# Autodesk Inventor assembly: STEEL FRAME ASSY
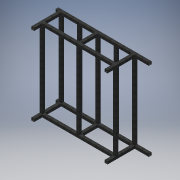
[picture p0: Inventor's stored thumbnail of the model, 180x180]
Saved by Autodesk Inventor 2017 (Build 210142000, 142)
## iProperties
Part Number: STEEL FRAME ASSY
Material: Genérico
Document SubType Name: Assembly
Designer: Cristian
Author: Cristian
## Documents named in this file (6)
- C:\Users\Cristian\Desktop\DISEÑO\FRAME\CNCO 75-3 FRAME\STEEL FRAME ASSY.iam
- C:\Users\Cristian\Desktop\DISEÑO\FRAME\CNCO 75-3 FRAME\2570 STEEL PROFILE.ipt
- C:\Users\Cristian\Desktop\DISEÑO\FRAME\CNCO 75-3 FRAME\2100 STEEL PROFILE.ipt
- C:\Users\Cristian\Desktop\DISEÑO\FRAME\CNCO 75-3 FRAME\450 STEEL PROFILE.ipt
- C:\Users\Cristian\Desktop\DISEÑO\FRAME\CNCO 75-3 FRAME\750 STEEL PROFILE.ipt
- C:\Users\Cristian\Desktop\DISEÑO\FRAME\CNCO 75-3 FRAME\1950 STEEL PROFILE.ipt
## Components (18 placed, 5 different names)
1. 2100 STEEL PROFILE:1 — Coincidencia:1, Coincidencia:2, Coincidencia:3, Coincidencia:4, Nivelación:1, Coincidencia:5, Nivelación:2, Nivelación:3, Nivelación:6, Nivelación:21, Nivelación:23
2. 2570 STEEL PROFILE:1 — Coincidencia:4, Nivelación:1, Coincidencia:6, Nivelación:4, Coincidencia:9, Nivelación:9, Nivelación:10, Coincidencia:16, Nivelación:14, Nivelación:18
3. 2570 STEEL PROFILE:2 — Coincidencia:5, Nivelación:2, Coincidencia:7, Nivelación:5, Coincidencia:8, Nivelación:7, Nivelación:8, Coincidencia:14, Nivelación:13, Coincidencia:18, Nivelación:15, Coincidencia:19, Nivelación:19, Coincidencia:20, Nivelación:22, Coincidencia:21, Nivelación:24
4. 450 STEEL PROFILE:1 — Coincidencia:6, Nivelación:3, Nivelación:4, Coincidencia:13
5. 450 STEEL PROFILE:2 — Coincidencia:7, Nivelación:5, Nivelación:6, Coincidencia:11, Nivelación:31
6. 750 STEEL PROFILE:1 — Coincidencia:16, Nivelación:14, Coincidencia:17
7. 750 STEEL PROFILE:2 — Coincidencia:14, Nivelación:13, Coincidencia:15, Nivelación:20, Coincidencia:23, Nivelación:28
8. 750 STEEL PROFILE:3 — Coincidencia:8, Nivelación:7, Nivelación:8, Coincidencia:10, Nivelación:11, Nivelación:16, Coincidencia:22, Nivelación:27
9. 750 STEEL PROFILE:4 — Coincidencia:9, Nivelación:9, Nivelación:10, Coincidencia:12, Nivelación:12, Nivelación:17
10. 1950 STEEL PROFILE:1 — Coincidencia:10, Nivelación:11, Coincidencia:11, Coincidencia:15, Nivelación:26, Nivelación:29, Coincidencia:24, Nivelación:30
11. 1950 STEEL PROFILE:2 — Coincidencia:12, Nivelación:12, Coincidencia:13, Coincidencia:17
12. 2100 STEEL PROFILE:2 — Coincidencia:21, Nivelación:24, Nivelación:25
13. 2100 STEEL PROFILE:3 — Coincidencia:20, Nivelación:22, Nivelación:23
14. 2100 STEEL PROFILE:4 — Coincidencia:18, Nivelación:15, Nivelación:16, Nivelación:17, Nivelación:18, Nivelación:25
15. 2100 STEEL PROFILE:5 — Coincidencia:19, Nivelación:19, Nivelación:20, Nivelación:21
16. 2100 STEEL PROFILE:6 — Coincidencia:22, Nivelación:26, Nivelación:27
17. 2100 STEEL PROFILE:7 — Coincidencia:23, Nivelación:28, Nivelación:29
18. 2100 STEEL PROFILE:8 — Coincidencia:24, Nivelación:30, Nivelación:31
## Relationships (55: Flush 31, Mate 24)
- Coincidencia:1 [Mate]: 2100 STEEL PROFILE:1
- Coincidencia:2 [Mate]: 2100 STEEL PROFILE:1
- Coincidencia:3 [Mate]: 2100 STEEL PROFILE:1
- Coincidencia:4 [Mate]: 2100 STEEL PROFILE:1 ↔ 2570 STEEL PROFILE:1
- Nivelación:1 [Flush]: 2100 STEEL PROFILE:1 ↔ 2570 STEEL PROFILE:1
- Coincidencia:5 [Mate]: 2100 STEEL PROFILE:1 ↔ 2570 STEEL PROFILE:2
- Nivelación:2 [Flush]: 2100 STEEL PROFILE:1 ↔ 2570 STEEL PROFILE:2
- Coincidencia:6 [Mate]: 2570 STEEL PROFILE:1 ↔ 450 STEEL PROFILE:1
- Nivelación:3 [Flush]: 2100 STEEL PROFILE:1 ↔ 450 STEEL PROFILE:1
- Nivelación:4 [Flush]: 2570 STEEL PROFILE:1 ↔ 450 STEEL PROFILE:1
- Coincidencia:7 [Mate]: 2570 STEEL PROFILE:2 ↔ 450 STEEL PROFILE:2
- Nivelación:5 [Flush]: 2570 STEEL PROFILE:2 ↔ 450 STEEL PROFILE:2
- Nivelación:6 [Flush]: 2100 STEEL PROFILE:1 ↔ 450 STEEL PROFILE:2
- Coincidencia:8 [Mate]: 2570 STEEL PROFILE:2 ↔ 750 STEEL PROFILE:3
- Nivelación:7 [Flush]: 2570 STEEL PROFILE:2 ↔ 750 STEEL PROFILE:3
- Nivelación:8 [Flush] (-390 mm): 2570 STEEL PROFILE:2 ↔ 750 STEEL PROFILE:3
- Coincidencia:9 [Mate]: 2570 STEEL PROFILE:1 ↔ 750 STEEL PROFILE:4
- Nivelación:9 [Flush]: 2570 STEEL PROFILE:1 ↔ 750 STEEL PROFILE:4
- Nivelación:10 [Flush] (390 mm): 2570 STEEL PROFILE:1 ↔ 750 STEEL PROFILE:4
- Coincidencia:10 [Mate]: 750 STEEL PROFILE:3 ↔ 1950 STEEL PROFILE:1
- Nivelación:11 [Flush]: 750 STEEL PROFILE:3 ↔ 1950 STEEL PROFILE:1
- Coincidencia:11 [Mate]: 450 STEEL PROFILE:2 ↔ 1950 STEEL PROFILE:1
- Coincidencia:12 [Mate]: 750 STEEL PROFILE:4 ↔ 1950 STEEL PROFILE:2
- Nivelación:12 [Flush]: 750 STEEL PROFILE:4 ↔ 1950 STEEL PROFILE:2
- Coincidencia:13 [Mate]: 450 STEEL PROFILE:1 ↔ 1950 STEEL PROFILE:2
- Coincidencia:14 [Mate]: 2570 STEEL PROFILE:2 ↔ 750 STEEL PROFILE:2
- Nivelación:13 [Flush]: 2570 STEEL PROFILE:2 ↔ 750 STEEL PROFILE:2
- Coincidencia:15 [Mate]: 750 STEEL PROFILE:2 ↔ 1950 STEEL PROFILE:1
- Coincidencia:16 [Mate]: 2570 STEEL PROFILE:1 ↔ 750 STEEL PROFILE:1
- Nivelación:14 [Flush]: 2570 STEEL PROFILE:1 ↔ 750 STEEL PROFILE:1
- Coincidencia:17 [Mate]: 750 STEEL PROFILE:1 ↔ 1950 STEEL PROFILE:2
- Coincidencia:18 [Mate]: 2570 STEEL PROFILE:2 ↔ 2100 STEEL PROFILE:4
- Nivelación:15 [Flush]: 2570 STEEL PROFILE:2 ↔ 2100 STEEL PROFILE:4
- Nivelación:16 [Flush]: 750 STEEL PROFILE:3 ↔ 2100 STEEL PROFILE:4
- Nivelación:17 [Flush]: 750 STEEL PROFILE:4 ↔ 2100 STEEL PROFILE:4
- Nivelación:18 [Flush]: 2570 STEEL PROFILE:1 ↔ 2100 STEEL PROFILE:4
- Coincidencia:19 [Mate]: 2570 STEEL PROFILE:2 ↔ 2100 STEEL PROFILE:5
- Nivelación:19 [Flush]: 2570 STEEL PROFILE:2 ↔ 2100 STEEL PROFILE:5
- Nivelación:20 [Flush]: 750 STEEL PROFILE:2 ↔ 2100 STEEL PROFILE:5
- Nivelación:21 [Flush] (1012.5 mm): 2100 STEEL PROFILE:1 ↔ 2100 STEEL PROFILE:5
- Coincidencia:20 [Mate]: 2570 STEEL PROFILE:2 ↔ 2100 STEEL PROFILE:3
- Nivelación:22 [Flush]: 2570 STEEL PROFILE:2 ↔ 2100 STEEL PROFILE:3
- Nivelación:23 [Flush] (506.25 mm): 2100 STEEL PROFILE:1 ↔ 2100 STEEL PROFILE:3
- Coincidencia:21 [Mate]: 2570 STEEL PROFILE:2 ↔ 2100 STEEL PROFILE:2
- Nivelación:24 [Flush]: 2570 STEEL PROFILE:2 ↔ 2100 STEEL PROFILE:2
- Nivelación:25 [Flush] (506.25 mm): 2100 STEEL PROFILE:2 ↔ 2100 STEEL PROFILE:4
- Coincidencia:22 [Mate]: 750 STEEL PROFILE:3 ↔ 2100 STEEL PROFILE:6
- Nivelación:26 [Flush]: 1950 STEEL PROFILE:1 ↔ 2100 STEEL PROFILE:6
- Nivelación:27 [Flush]: 750 STEEL PROFILE:3 ↔ 2100 STEEL PROFILE:6
- Coincidencia:23 [Mate]: 750 STEEL PROFILE:2 ↔ 2100 STEEL PROFILE:7
- Nivelación:28 [Flush]: 750 STEEL PROFILE:2 ↔ 2100 STEEL PROFILE:7
- Nivelación:29 [Flush]: 1950 STEEL PROFILE:1 ↔ 2100 STEEL PROFILE:7
- Coincidencia:24 [Mate]: 1950 STEEL PROFILE:1 ↔ 2100 STEEL PROFILE:8
- Nivelación:30 [Flush]: 1950 STEEL PROFILE:1 ↔ 2100 STEEL PROFILE:8
- Nivelación:31 [Flush]: 450 STEEL PROFILE:2 ↔ 2100 STEEL PROFILE:8
## Named parameters: length_t = 2100 mm, width_t = 2100 mm, size_p = 75 mm, voladizo = 390 mm
